# Autodesk Inventor assembly: ASY MSC 203 RIGHT BOARD
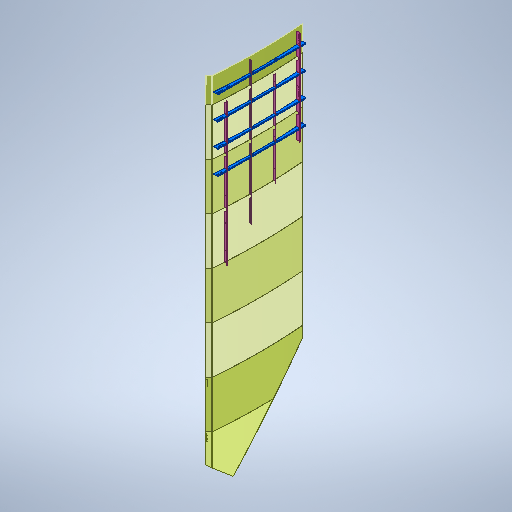
[picture p0: Inventor's stored thumbnail of the model, 512x512]
Saved by Autodesk Inventor 2025 (Build 290162010, 162A)
## iProperties
Created: 2024-07-22
Part Number: ASY MSC 203 RIGHT BOARD
Document SubType Name: Assembly
Designer: pokla
Author: pokla
## Documents named in this file (10)
- C:\Users\pokla\Documents\Inventor\Отстойник осветлитель\Manturovo_Se-clar-Gleb\ASY MSC 203 RIGHT BOARD.iam
- C:\Users\pokla\Documents\Inventor\Отстойник осветлитель\Manturovo_Se-clar-Gleb\MSC 052 rib board.ipt
- C:\Users\pokla\Documents\Inventor\Отстойник осветлитель\Manturovo_Se-clar-Gleb\MSC 024 sheet board main.ipt
- C:\Users\pokla\Documents\Inventor\Отстойник осветлитель\Manturovo_Se-clar-Gleb\MSC 023 sheet board.ipt
- C:\Users\pokla\Documents\Inventor\Отстойник осветлитель\Manturovo_Se-clar-Gleb\MSC 025.2 sheet board withers.ipt
- C:\Users\pokla\Documents\Inventor\Отстойник осветлитель\Manturovo_Se-clar-Gleb\MSC 063 stringer BOARD  #.ipt
- C:\Users\pokla\Documents\Inventor\Отстойник осветлитель\Manturovo_Se-clar-Gleb\MSC 064 stringer BOARD  ##.ipt
- C:\Users\pokla\Documents\Inventor\Отстойник осветлитель\Manturovo_Se-clar-Gleb\MSC 027.2 sheet board withers 4.ipt
- C:\Users\pokla\Documents\Inventor\Отстойник осветлитель\Manturovo_Se-clar-Gleb\MSC 065 stringer BOARD  ###.ipt
- C:\Users\pokla\Documents\Inventor\Отстойник осветлитель\Manturovo_Se-clar-Gleb\MSC 065 stringer BOARD  ####.ipt
## Components (22 placed, 10 different names)
1. MSC 023 sheet board.ipt:2 — Flush:2, Flush:3, Flush:4, Rigid:1, Flush:5, Angle:1, Tangent:1, Tangent:2
2. MSC 024 sheet board main.ipt:10 — Rigid:1, Rigid:2
3. MSC 024 sheet board main.ipt:9 — Rigid:2, Rigid:3
4. MSC 024 sheet board main.ipt:8 — Rigid:3, Rigid:4
5. MSC 024 sheet board main.ipt:7 — Rigid:4, Rigid:5
6. MSC 024 sheet board main.ipt:6 — Rigid:5, Rigid:19
7. MSC 025.2 sheet board withers:1 — Rigid:19, Rigid:20
8. MSC 027.2 sheet board withers 4:1 — Rigid:20
9. MSC 052 rib board.ipt:1 — Flush:5, Angle:1, Tangent:1, Tangent:2, Rigid:18
10. MSC 052 rib board.ipt:4 — Rigid:12, Rigid:15, Rigid:16, Rigid:17
11. MSC 052 rib board:3 — Rigid:13
12. MSC 063 stringer BOARD  #:1 — Rigid:6, Rigid:12, Rigid:18
13. MSC 064 stringer BOARD  ##:1 — Rigid:7, Rigid:16
14. MSC 065 stringer BOARD  ###:1 — Rigid:8, Rigid:9
15. MSC 065 stringer BOARD  ####:1 — Rigid:10, Rigid:11
16. MSC 065 stringer BOARD  ####:2 — Rigid:10, Rigid:15
17. MSC 065 stringer BOARD  ###:2 — Rigid:8, Rigid:17
18. MSC 063 stringer BOARD  #:2 — Rigid:6, Rigid:13, Rigid:14
19. MSC 064 stringer BOARD  ##:2 — Rigid:7
20. MSC 065 stringer BOARD  ###:3 — Rigid:9
21. MSC 065 stringer BOARD  ####:3 — Rigid:11
22. MSC 052 rib board:5 — Rigid:14
## Relationships (27: WeldJoint 20, Flush 4, Tangent 2, Angle 1)
- Flush:2: MSC 023 sheet board.ipt:2
- Flush:3: MSC 023 sheet board.ipt:2
- Flush:4: MSC 023 sheet board.ipt:2
- Rigid:1 [WeldJoint]: MSC 023 sheet board.ipt:2 ↔ MSC 024 sheet board main.ipt:10
- Rigid:2 [WeldJoint]: MSC 024 sheet board main.ipt:10 ↔ MSC 024 sheet board main.ipt:9
- Rigid:3 [WeldJoint]: MSC 024 sheet board main.ipt:9 ↔ MSC 024 sheet board main.ipt:8
- Rigid:4 [WeldJoint]: MSC 024 sheet board main.ipt:8 ↔ MSC 024 sheet board main.ipt:7
- Rigid:5 [WeldJoint]: MSC 024 sheet board main.ipt:7 ↔ MSC 024 sheet board main.ipt:6
- Flush:5 (304 mm): MSC 023 sheet board.ipt:2 ↔ MSC 052 rib board.ipt:1
- Angle:1 (0 deg): MSC 023 sheet board.ipt:2 ↔ MSC 052 rib board.ipt:1
- Tangent:1: MSC 023 sheet board.ipt:2 ↔ MSC 052 rib board.ipt:1
- Tangent:2: MSC 023 sheet board.ipt:2 ↔ MSC 052 rib board.ipt:1
- Rigid:6 [WeldJoint]: MSC 063 stringer BOARD  #:1 ↔ MSC 063 stringer BOARD  #:2
- Rigid:7 [WeldJoint]: MSC 064 stringer BOARD  ##:1 ↔ MSC 064 stringer BOARD  ##:2
- Rigid:8 [WeldJoint]: MSC 065 stringer BOARD  ###:1 ↔ MSC 065 stringer BOARD  ###:2
- Rigid:9 [WeldJoint]: MSC 065 stringer BOARD  ###:1 ↔ MSC 065 stringer BOARD  ###:3
- Rigid:10 [WeldJoint]: MSC 065 stringer BOARD  ####:1 ↔ MSC 065 stringer BOARD  ####:2
- Rigid:11 [WeldJoint]: MSC 065 stringer BOARD  ####:1 ↔ MSC 065 stringer BOARD  ####:3
- Rigid:12 [WeldJoint] (2 mm): MSC 052 rib board.ipt:4 ↔ MSC 063 stringer BOARD  #:1
- Rigid:13 [WeldJoint] (2 mm): MSC 052 rib board:3 ↔ MSC 063 stringer BOARD  #:2
- Rigid:14 [WeldJoint] (2 mm): MSC 063 stringer BOARD  #:2 ↔ MSC 052 rib board:5
- Rigid:15 [WeldJoint] (2 mm): MSC 052 rib board.ipt:4 ↔ MSC 065 stringer BOARD  ####:2
- Rigid:16 [WeldJoint] (2 mm): MSC 052 rib board.ipt:4 ↔ MSC 064 stringer BOARD  ##:1
- Rigid:17 [WeldJoint] (2 mm): MSC 052 rib board.ipt:4 ↔ MSC 065 stringer BOARD  ###:2
- Rigid:18 [WeldJoint] (2 mm): MSC 052 rib board.ipt:1 ↔ MSC 063 stringer BOARD  #:1
- Rigid:19 [WeldJoint]: MSC 024 sheet board main.ipt:6 ↔ MSC 025.2 sheet board withers:1
- Rigid:20 [WeldJoint]: MSC 025.2 sheet board withers:1 ↔ MSC 027.2 sheet board withers 4:1
